# Autodesk Inventor assembly: ASY МОО 001 отстойник осветлитель
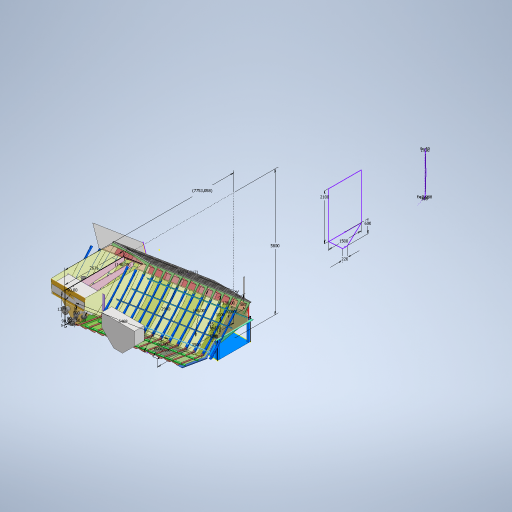
[picture p0: Inventor's stored thumbnail of the model, 512x512]
Saved by Autodesk Inventor 2024.2 (Build 282272000, 272)
## iProperties
Created: 2024-04-28
Part Number: ASY МОО 001 отстойник осветлитель
Document SubType Name: Weldment
Designer: admin
Weld Material: Welded Aluminum-6061
Mass: 1.58517e+06 g
Surface Area: 1.48953e+06 cm^2
Volume: 226523 cm^3
Density: 6.99781 g/cm^3
Author: admin
## Documents named in this file (52)
- C:\Users\admin\YandexDisk-badmisterfox\домашниий пк\Inventor\Manturovo\Manturovo_Se-clar\ASY МОО 001 отстойник осветлитель.iam
- C:\Users\admin\YandexDisk-badmisterfox\домашниий пк\Inventor\Manturovo\Manturovo_Se-clar\МОО 033 лист спина базовый.ipt
- C:\Users\admin\YandexDisk-badmisterfox\домашниий пк\Inventor\Manturovo\Manturovo_Se-clar\Пример емкости.ipt
- C:\Users\admin\YandexDisk-badmisterfox\домашниий пк\Inventor\Manturovo\Manturovo_Se-clar\МОО 041 лист брюхо основной.ipt
- C:\Users\admin\YandexDisk-badmisterfox\домашниий пк\Inventor\Manturovo\Manturovo_Se-clar\МОО 052 шпангоут борт.ipt
- C:\Users\admin\YandexDisk-badmisterfox\домашниий пк\Inventor\Manturovo\Manturovo_Se-clar\МОО 051 шпангоут спина.ipt
- C:\Users\admin\YandexDisk-badmisterfox\домашниий пк\Inventor\Manturovo\Manturovo_Se-clar\Рама основания\ASY МОО 040 рама основания.iam
- C:\Users\admin\YandexDisk-badmisterfox\домашниий пк\Inventor\Manturovo\Manturovo_Se-clar\ASY МОО 060 ракета.iam
- C:\Users\admin\YandexDisk-badmisterfox\домашниий пк\Inventor\Manturovo\Manturovo_Se-clar\Content Center Files\en-US\ISO 5251 B 3D\ISO 5251 Bends 3D without straight ends(90 deg) DN80 2 2.ipt
- C:\Users\admin\YandexDisk-badmisterfox\домашниий пк\Inventor\Manturovo\Manturovo_Se-clar\Content Center Files\en-US\ISO 5251(1)\ISO 5251 Concentric reducers DN80 x DN65 3,2 3,2.ipt
- C:\Users\admin\YandexDisk-badmisterfox\домашниий пк\Inventor\Manturovo\Manturovo_Se-clar\ASY МОО 010 конус.iam
- C:\Users\admin\YandexDisk-badmisterfox\домашниий пк\Inventor\Manturovo\Manturovo_Se-clar\ракета\МОО 064 ракета труба.ipt
- C:\Users\admin\YandexDisk-badmisterfox\домашниий пк\Inventor\Manturovo\Manturovo_Se-clar\х_размеры МОО отстойник осветлитель Dummu.ipt
- C:\Users\admin\YandexDisk-badmisterfox\домашниий пк\Inventor\Manturovo\Manturovo_Se-clar\МОО 031 лист спина поясница.ipt
- C:\Users\admin\YandexDisk-badmisterfox\домашниий пк\Inventor\Manturovo\Manturovo_Se-clar\Content Center Files\en-US\DIN EN 1092-1 01 - PN 25\DIN EN 1092-1 Plate Flange for Welding Type 01 - PN 25 80 x 88.9.ipt
- C:\Users\admin\YandexDisk-badmisterfox\домашниий пк\Inventor\Manturovo\Manturovo_Se-clar\МОО 024 лист борт основной.ipt
- C:\Users\admin\YandexDisk-badmisterfox\домашниий пк\Inventor\Manturovo\Manturovo_Se-clar\МОО 032 лист спина-поясница магич.ipt
- C:\Users\admin\YandexDisk-badmisterfox\домашниий пк\Inventor\Manturovo\Manturovo_Se-clar\МОО 021 лист левый борт бедро.ipt
- C:\Users\admin\YandexDisk-badmisterfox\домашниий пк\Inventor\Manturovo\Manturovo_Se-clar\МОО 022 лист правый борт бедро.ipt
- C:\Users\admin\YandexDisk-badmisterfox\домашниий пк\Inventor\Manturovo\Manturovo_Se-clar\МОО 034 лист спина-холка.ipt
- C:\Users\admin\YandexDisk-badmisterfox\домашниий пк\Inventor\Manturovo\Manturovo_Se-clar\МОО 042 лист брюхо-горло.ipt
- C:\Users\admin\YandexDisk-badmisterfox\домашниий пк\Inventor\Manturovo\Manturovo_Se-clar\МОО 023 лист борт.ipt
- C:\Users\admin\YandexDisk-badmisterfox\домашниий пк\Inventor\Manturovo\Manturovo_Se-clar\конус\МОО 071 гребень 1.ipt
- C:\Users\admin\YandexDisk-badmisterfox\домашниий пк\Inventor\Manturovo\Manturovo_Se-clar\конус\МОО 072 гребень 2.ipt
- C:\Users\admin\YandexDisk-badmisterfox\домашниий пк\Inventor\Manturovo\Manturovo_Se-clar\конус\МОО 073 морда 3.ipt
- C:\Users\admin\YandexDisk-badmisterfox\домашниий пк\Inventor\Manturovo\Manturovo_Se-clar\Content Center Files\en-US\ISO 5251 B 3D\ISO 5251 Bends 3D without straight ends(90 deg) DN150 11 11.ipt
- C:\Users\admin\YandexDisk-badmisterfox\домашниий пк\Inventor\Manturovo\Manturovo_Se-clar\Content Center Files\en-US\DIN EN 1092-1 01 - PN 25\DIN EN 1092-1 Plate Flange for Welding Type 01 - PN 25 150 x 168.3.ipt
- C:\Users\admin\YandexDisk-badmisterfox\домашниий пк\Inventor\Manturovo\Manturovo_Se-clar\МОО 061 труба верх 1.ipt
- C:\Users\admin\YandexDisk-badmisterfox\домашниий пк\Inventor\Manturovo\Manturovo_Se-clar\МОО 062 труба верх 2.ipt
- C:\Users\admin\YandexDisk-badmisterfox\домашниий пк\Inventor\Manturovo\Manturovo_Se-clar\МОО 063 труба верх 3.ipt
- C:\Users\admin\YandexDisk-badmisterfox\домашниий пк\Inventor\Manturovo\Manturovo_Se-clar\МОО 061 стрингер спина ^.ipt
- C:\Users\admin\YandexDisk-badmisterfox\домашниий пк\Inventor\Manturovo\Manturovo_Se-clar\МОО 063 стрингер борт #.ipt
- C:\Users\admin\YandexDisk-badmisterfox\домашниий пк\Inventor\Manturovo\Manturovo_Se-clar\МОО 062 стрингер спина ^^.ipt
- C:\Users\admin\YandexDisk-badmisterfox\домашниий пк\Inventor\Manturovo\Manturovo_Se-clar\МОО 064 стрингер борт ##.ipt
- C:\Users\admin\YandexDisk-badmisterfox\домашниий пк\Inventor\Manturovo\Manturovo_Se-clar\МОО 065 стрингер борт ###.ipt
- C:\Users\admin\YandexDisk-badmisterfox\домашниий пк\Inventor\Manturovo\Manturovo_Se-clar\МОО 066 стрингер борт ####.ipt
- C:\Users\admin\YandexDisk-badmisterfox\домашниий пк\Inventor\Manturovo\Manturovo_Se-clar\МОО 067 стрингер борт живот.ipt
- C:\Users\admin\YandexDisk-badmisterfox\домашниий пк\Inventor\Manturovo\Manturovo_Se-clar\МОО 053 шпангоут брюхо.ipt
- C:\Users\admin\YandexDisk-badmisterfox\домашниий пк\Inventor\Manturovo\Manturovo_Se-clar\МОО 025 лист борт холка.ipt
- C:\Users\admin\YandexDisk-badmisterfox\домашниий пк\Inventor\Manturovo\Manturovo_Se-clar\МОО 026 лист борт морда.ipt
- C:\Users\admin\YandexDisk-badmisterfox\домашниий пк\Inventor\Manturovo\Manturovo_Se-clar\Part1.ipt
- C:\Users\admin\YandexDisk-badmisterfox\домашниий пк\Inventor\Manturovo\Manturovo_Se-clar\стапель\ASY стапель.iam
- C:\Users\admin\YandexDisk-badmisterfox\домашниий пк\Inventor\Manturovo\Manturovo_Se-clar\DXF файлы\Шпангоуты+стрингеры\МОО 0100.ipt
- C:\Users\admin\YandexDisk-badmisterfox\домашниий пк\Inventor\Manturovo\Manturovo_Se-clar\МОО 025 лист борт холка_MIR.ipt
- C:\Users\admin\YandexDisk-badmisterfox\домашниий пк\Inventor\Manturovo\Manturovo_Se-clar\МОО 026 лист борт морда_MIR.ipt
- C:\Users\admin\YandexDisk-badmisterfox\домашниий пк\Inventor\Manturovo\Manturovo_Se-clar\МОО 068 stringer lowerback.ipt
- C:\Users\admin\YandexDisk-badmisterfox\домашниий пк\Inventor\Manturovo\Manturovo_Se-clar\конус\МОО 071 гребень 1_MIR.ipt
- C:\Users\admin\YandexDisk-badmisterfox\домашниий пк\Inventor\Manturovo\Manturovo_Se-clar\Для удаления\DUMMY 2.ipt
- C:\Users\admin\YandexDisk-badmisterfox\домашниий пк\Inventor\Manturovo\Manturovo_Se-clar\MSC 075 face 5.ipt
- C:\Users\admin\YandexDisk-badmisterfox\домашниий пк\Inventor\Manturovo\Manturovo_Se-clar\MSC 075 face 6.ipt
- C:\Users\admin\YandexDisk-badmisterfox\домашниий пк\Inventor\Manturovo\Manturovo_Se-clar\Для удаления\DUMMY 3.ipt
- C:\Users\admin\YandexDisk-badmisterfox\домашниий пк\Inventor\Manturovo\Manturovo_Se-clar\MSC 077 face 7.ipt
## Components (212 placed, 64 different names)
1. Пример емкости.ipt:1 — Mate:1, Mate:2, Flush:2
2. х_размеры МОО отстойник осветлитель Dummu.ipt:1
3. ASY МОО 040 рама основания.iam:1 [sub-assembly] — Flush:19, Flush:20, Flush:21
4. МОО 033 лист спина базовый.ipt:1 — Flush:3, Rigid:11, Rigid:12
5. МОО 041 лист брюхо основной.ipt:1 — Mate:9, Rigid:18, Rigid:40
6. ASY МОО 060 ракета.iam:1 [sub-assembly] — Flush:23, Rigid:10
7. ISO 5251 Bends 3D without straight ends(90 deg) DN80 2 2.ipt:1 — Rigid:2, Rigid:3
8. ISO 5251 Concentric reducers DN80 x DN65 3,2 3,2.ipt:1 — Rigid:2, Rigid:10
9. ASY МОО 010 конус.iam:1 [sub-assembly] — Flush:22, Mate:16, Flush:28, Mate:31, Mate:36, Mate:54, Mate:57, Mate:65
10. МОО 064 ракета труба.ipt:1 — Rigid:3, Cylindrical:1
11. МОО 033 лист спина базовый.ipt:2 — Rigid:11, Tangent:1, Tangent:3, Rigid:37
12. МОО 033 лист спина базовый.ipt:3 — Flush:24, Rigid:12, Mate:19, Mate:22, Rigid:30, Mate:31, Flush:44, Tangent:8, Tangent:9
13. МОО 031 лист спина поясница.ipt:1 — Mate:15, Mate:16, Flush:27, Mate:19, Mate:22, Tangent:10
14. DIN EN 1092-1 Plate Flange for Welding Type 01 - PN 25 80 x 88.9.ipt:1 — Flush:25, Flush:26, Mate:18, Cylindrical:1
15. МОО 024 лист борт основной.ipt:1 — Flush:30, Tangent:1, Rigid:35, Mate:37
16. МОО 041 лист брюхо основной.ipt:2 — Rigid:18, Rigid:53
17. МОО 032 лист спина-поясница магич.ipt:1 — Mate:24, Rigid:30, Flush:42, Tangent:6, Flush:43, Tangent:7
18. МОО 021 лист левый борт бедро.ipt:1 — Flush:41, Flush:42, Tangent:6
19. МОО 022 лист правый борт бедро.ipt:1 — Mate:30, Flush:43, Tangent:7
20. МОО 024 лист борт основной.ipt:2 — Rigid:35, Rigid:36
21. МОО 024 лист борт основной.ipt:3 — Rigid:36, Rigid:49
22. МОО 033 лист спина базовый.ipt:4 — Rigid:37, Rigid:38
23. МОО 033 лист спина базовый.ipt:5 — Rigid:38, Rigid:39
24. МОО 034 лист спина-холка.ipt:1 — Rigid:39
25. МОО 041 лист брюхо основной.ipt:3 — Rigid:40, Rigid:47
26. МОО 042 лист брюхо-горло.ipt:1 — Rigid:48, Mate:70, Mate:71
27. МОО 041 лист брюхо основной.ipt:4 — Rigid:45, Rigid:47
28. МОО 041 лист брюхо основной.ipt:5 — Rigid:45, Rigid:48
29. МОО 024 лист борт основной.ipt:4 — Rigid:49, Rigid:50
30. МОО 024 лист борт основной.ipt:5 — Rigid:50, Rigid:113
31. МОО 023 лист борт.ipt:1 — Mate:36, Flush:47, Tangent:8, Mate:37, Mate:55
32. МОО 071 гребень 1.ipt:1 — Mate:50, Flush:57, Mate:68
33. МОО 073 морда 3.ipt:2 — Rigid:156, Rigid:157, Mate:70, Flush:62, Mate:71, Rigid:159
34. МОО 041 лист брюхо основной.ipt:6 — Mate:54, Mate:55, Rigid:53
35. DIN EN 1092-1 Plate Flange for Welding Type 01 - PN 25 80 x 88.9.ipt:2 — Rigid:62
36. МОО 072 гребень 2.ipt:2 — Flush:56, Flush:57, Mate:68, Flush:59, Mate:77, Flush:78
37. DIN EN 1092-1 Plate Flange for Welding Type 01 - PN 25 150 x 168.3.ipt:1 — Rigid:158
38. МОО 061 труба верх 1.ipt:1 — Rigid:158, Rigid:59, Rigid:159
39. ISO 5251 Bends 3D without straight ends(90 deg) DN150 11 11.ipt:1 — Rigid:59, Rotational:2
40. МОО 062 труба верх 2.ipt:1 — Rigid:132, Rigid:156
41. DIN EN 1092-1 Plate Flange for Welding Type 01 - PN 25 150 x 168.3.ipt:2 — Rigid:132
42. МОО 063 труба верх 3.ipt:1 — Rigid:62, Rigid:157
43. МОО 024 лист борт основной.ipt:6 — Rigid:134
44. МОО 024 лист борт основной.ipt:7
45. МОО 024 лист борт основной.ipt:8
46. МОО 024 лист борт основной.ipt:9
47. МОО 024 лист борт основной.ipt:10 — Rigid:67
48. МОО 023 лист борт.ipt:2 — Rigid:67, Mate:57, Mate:58, Tangent:9
49. МОО 052 шпангоут борт.ipt:1 — Rigid:74, Rigid:128, Rigid:129
50. МОО 051 шпангоут спина.ipt:1 — Rigid:25, Rigid:74, Rigid:91, Rigid:93, Rigid:139
51. МОО 066 стрингер борт ####.ipt:1 — Rigid:143
52. МОО 065 стрингер борт ###.ipt:1 — Rigid:142
53. МОО 064 стрингер борт ##.ipt:1 — Rigid:129, Rigid:141
54. МОО 063 стрингер борт #.ipt:1 — Rigid:128, Rigid:140
55. МОО 062 стрингер спина ^^.ipt:1 — Rigid:93, Rigid:155
56. МОО 061 стрингер спина ^.ipt:2 — Rigid:91, Rigid:153
57. МОО 061 стрингер спина ^.ipt:1 — Rigid:90, Rigid:152
58. МОО 025 лист борт холка.ipt:1 — Rigid:113, Rigid:114
59. МОО 026 лист борт морда.ipt:1 — Rigid:114, Flush:56, Mate:69, Flush:60, Mate:75
60. Part1.ipt:1
61. МОО 051 шпангоут спина.ipt:2 — Rigid:116, Rigid:121, Rigid:130, Rigid:131
62. МОО 051 шпангоут спина.ipt:3 — Rigid:116
63. МОО 051 шпангоут спина.ipt:4 — Rigid:131
64. МОО 051 шпангоут спина.ipt:5 — Mate:62, Flush:53
65. МОО 052 шпангоут борт.ipt:2 — Rigid:121
66. МОО 062 стрингер спина ^^.ipt:2 — Rigid:92, Mate:66, Rigid:154
67. МОО 066 стрингер борт ####.ipt:2 — Rigid:125, Rigid:151
68. МОО 063 стрингер борт #.ipt:2 — Rigid:122, Rigid:148
69. МОО 064 стрингер борт ##.ipt:2 — Rigid:123, Rigid:149
70. МОО 065 стрингер борт ###.ipt:2 — Rigid:124, Rigid:150
71. МОО 052 шпангоут борт.ipt:3 — Rigid:72, Rigid:122, Rigid:123, Flush:51, Flush:52, Rigid:124, Rigid:125, Mate:61
72. МОО 051 шпангоут спина.ipt:6 — Flush:12, Tangent:3, Rigid:25, Flush:44, Rigid:72, Rigid:90, Rigid:92, Rigid:130
73. ASY стапель.iam:1 [sub-assembly] — Mate:62, Flush:53, Mate:63
74. МОО 053 шпангоут брюхо.ipt:2 — Rigid:110, Flush:51, Flush:52, Rigid:126, Mate:61, Rigid:127
75. МОО 053 шпангоут брюхо.ipt:1 — Rigid:111, Rigid:112, Rigid:127
76. МОО 067 стрингер борт живот.ipt:4 — Rigid:126, Rigid:147
77. МОО 067 стрингер борт живот.ipt:3 — Rigid:110, Rigid:146
78. МОО 067 стрингер борт живот.ipt:2 — Rigid:112, Rigid:144
79. МОО 067 стрингер борт живот.ipt:1 — Rigid:111, Rigid:145
80. МОО 0100.ipt:1 — Mate:64
81. МОО 025 лист борт холка_MIR:1 — Rigid:133, Rigid:134
82. МОО 026 лист борт морда_MIR:1 — Rigid:133
83. МОО 068 stringer lowerback:1 — Mate:65, Mate:66, Tangent:10
84. МОО 071 гребень 1_MIR:1 — Flush:58
85. МОО 061 труба верх 1:2 — Rotational:2
86. DUMMY 2:1 — Flush:59
87. MSC 075 face 5:1 — Mate:69, Flush:60, Flush:61, Mate:76
88. MSC 075 face 6:1 — Flush:76, Mate:75, Mate:76
89. DUMMY 3:1
90. DIN EN 1092-1 Plate Flange for Welding Type 01 - PN 25 80 x 88.9:3
91. МОО 063 труба верх 3:2
92. MSC 077 face 7:1 — Mate:77, Flush:77, Flush:78
93. МОО 042 шпангоут брюхо:4
94. МОО 052 шпангоут борт:5
95. МОО 051 шпангоут спина:31 — Rigid:139
96. МОО 051 шпангоут спина:30
97. МОО 052 шпангоут борт:4
98. МОО 042 шпангоут брюхо:3
99. МОО 042 шпангоут брюхо:5
100. МОО 052 шпангоут борт:6
101. МОО 051 шпангоут спина:32
102. МОО 051 шпангоут спина:33
103. МОО 052 шпангоут борт:7
104. МОО 042 шпангоут брюхо:6
105. МОО 042 шпангоут брюхо:7
106. МОО 052 шпангоут борт:8
107. МОО 051 шпангоут спина:34
108. МОО 051 шпангоут спина:35
109. МОО 052 шпангоут борт:9
110. МОО 042 шпангоут брюхо:8
111. МОО 042 шпангоут брюхо:9
112. МОО 052 шпангоут борт:10
113. МОО 051 шпангоут спина:36
114. МОО 051 шпангоут спина:37
115. МОО 052 шпангоут борт:11
116. МОО 042 шпангоут брюхо:10
117. МОО 042 шпангоут брюхо:11
118. МОО 052 шпангоут борт:12
119. МОО 051 шпангоут спина:38
120. МОО 051 шпангоут спина:39
121. МОО 052 шпангоут борт:13
122. МОО 042 шпангоут брюхо:12
123. МОО 042 шпангоут брюхо:13
124. МОО 052 шпангоут борт:14
125. МОО 051 шпангоут спина:40
126. МОО 051 шпангоут спина:41
127. МОО 052 шпангоут борт:15
128. МОО 042 шпангоут брюхо:14
129. МОО 042 шпангоут брюхо:15
130. МОО 052 шпангоут борт:16
131. МОО 051 шпангоут спина:42
132. МОО 051 шпангоут спина:43
133. МОО 052 шпангоут борт:17
134. МОО 042 шпангоут брюхо:16
135. МОО 042 шпангоут брюхо:17
136. МОО 052 шпангоут борт:18
137. МОО 051 шпангоут спина:44
138. МОО 051 шпангоут спина:45
139. МОО 052 шпангоут борт:19
140. МОО 042 шпангоут брюхо:18
141. МОО 042 шпангоут брюхо:19
142. МОО 052 шпангоут борт:20
143. МОО 051 шпангоут спина:46
144. МОО 051 шпангоут спина:47
145. МОО 052 шпангоут борт:21
146. МОО 042 шпангоут брюхо:20
147. МОО 042 шпангоут брюхо:21
148. МОО 052 шпангоут борт:22
149. МОО 051 шпангоут спина:48
150. МОО 051 шпангоут спина:49
151. МОО 052 шпангоут борт:23
152. МОО 042 шпангоут брюхо:22
153. МОО 042 шпангоут брюхо:23
154. МОО 052 шпангоут борт:24
155. МОО 051 шпангоут спина:50
156. МОО 051 шпангоут спина:51
157. МОО 052 шпангоут борт:25
158. МОО 042 шпангоут брюхо:24
159. МОО 042 шпангоут брюхо:25
160. МОО 052 шпангоут борт:26
161. МОО 051 шпангоут спина:52
162. МОО 051 шпангоут спина:53
163. МОО 052 шпангоут борт:27
164. МОО 042 шпангоут брюхо:26
165. МОО 053 стрингер борт 3:4 — Rigid:148
166. МОО 054 стрингер борт 4:4 — Rigid:149
167. МОО 055 стрингер борт 5:4 — Rigid:150
168. МОО 056 стрингер борт 6:4 — Rigid:151
169. МОО 057 стрингер борт 7:5 — Rigid:147
170. МОО 057 стрингер борт 7:6 — Rigid:146
171. МОО 052 стрингер спина 2:4 — Rigid:154
172. МОО 051 стрингер спина 1:4 — Rigid:152
173. МОО 051 стрингер спина 1:3 — Rigid:153
174. МОО 052 стрингер спина 2:3 — Rigid:155
175. МОО 053 стрингер борт 3:3 — Rigid:140
176. МОО 054 стрингер борт 4:3 — Rigid:141
177. МОО 055 стрингер борт 5:3 — Rigid:142
178. МОО 056 стрингер борт 6:3 — Rigid:143
179. МОО 057 стрингер борт 7:10 — Rigid:145
180. МОО 057 стрингер борт 7:9 — Rigid:144
181. МОО 053 стрингер борт 3:5
182. МОО 054 стрингер борт 4:5
183. МОО 055 стрингер борт 5:5
184. МОО 056 стрингер борт 6:5
185. МОО 057 стрингер борт 7:11
186. МОО 057 стрингер борт 7:12
187. МОО 052 стрингер спина 2:5
188. МОО 051 стрингер спина 1:5
189. МОО 051 стрингер спина 1:7
190. МОО 052 стрингер спина 2:7
191. МОО 053 стрингер борт 3:7
192. МОО 054 стрингер борт 4:7
193. МОО 055 стрингер борт 5:7
194. МОО 056 стрингер борт 6:7
195. МОО 057 стрингер борт 7:15
196. МОО 057 стрингер борт 7:17
197. МОО 053 стрингер борт 3:6
198. МОО 054 стрингер борт 4:6
199. МОО 055 стрингер борт 5:6
200. МОО 056 стрингер борт 6:6
201. МОО 057 стрингер борт 7:13
202. МОО 057 стрингер борт 7:14
203. МОО 052 стрингер спина 2:6
204. МОО 051 стрингер спина 1:6
205. МОО 051 стрингер спина 1:8
206. МОО 052 стрингер спина 2:8
207. МОО 053 стрингер борт 3:8
208. МОО 054 стрингер борт 4:8
209. МОО 055 стрингер борт 5:8
210. МОО 056 стрингер борт 6:8
211. МОО 057 стрингер борт 7:16
212. МОО 057 стрингер борт 7:18
## Component patterns: (12 elements, first: МОО 042 шпангоут брюхо:4 + МОО 052 шпангоут борт:5 + МОО 051 шпангоут спина:31 + МОО 051 шпангоут спина:30 + МОО 052 шпангоут борт:4 + МОО 042 шпангоут брюхо:3), (3 elements, first: МОО 053 стрингер борт 3:4 + МОО 054 стрингер борт 4:4 + МОО 055 стрингер борт 5:4 + МОО 056 стрингер борт 6:4 + МОО 057 стрингер борт 7:5 + МОО 057 стрингер борт 7:6 + МОО 052 стрингер спина 2:4 + МОО 051 стрингер спина 1:4 + МОО 051 стрингер спина 1:3 + МОО 052 стрингер спина 2:3 + МОО 053 стрингер борт 3:3 + МОО 054 стрингер борт 4:3 + МОО 055 стрингер борт 5:3 + МОО 056 стрингер борт 6:3 + МОО 057 стрингер борт 7:10 + МОО 057 стрингер борт 7:9)
## Relationships (155: WeldJoint 80, Flush 34, Mate 32, Tangent 7, CylindricalJoint 1, RevoluteJoint 1)
- Mate:1: Пример емкости.ipt:1
- Mate:2: Пример емкости.ipt:1
- Flush:2: Пример емкости.ipt:1
- Flush:3: МОО 033 лист спина базовый.ipt:1
- Mate:9: МОО 041 лист брюхо основной.ipt:1
- Flush:12: МОО 051 шпангоут спина.ipt:6
- Rigid:2 [WeldJoint]: ISO 5251 Bends 3D without straight ends(90 deg) DN80 2 2.ipt:1 ↔ ISO 5251 Concentric reducers DN80 x DN65 3,2 3,2.ipt:1
- Rigid:3 [WeldJoint]: ISO 5251 Bends 3D without straight ends(90 deg) DN80 2 2.ipt:1 ↔ МОО 064 ракета труба.ipt:1
- Flush:19 (-250 mm): ASY МОО 040 рама основания.iam:1
- Flush:20: ASY МОО 040 рама основания.iam:1
- Flush:21: ASY МОО 040 рама основания.iam:1
- Flush:22: ASY МОО 010 конус.iam:1
- Flush:23: ASY МОО 060 ракета.iam:1
- Mate:15: МОО 031 лист спина поясница.ipt:1
- Flush:24: МОО 033 лист спина базовый.ipt:3
- Mate:16: ASY МОО 010 конус.iam:1 ↔ МОО 031 лист спина поясница.ipt:1
- Flush:25: DIN EN 1092-1 Plate Flange for Welding Type 01 - PN 25 80 x 88.9.ipt:1
- Flush:26: DIN EN 1092-1 Plate Flange for Welding Type 01 - PN 25 80 x 88.9.ipt:1
- Mate:18 (120 mm): DIN EN 1092-1 Plate Flange for Welding Type 01 - PN 25 80 x 88.9.ipt:1
- Rigid:10 [WeldJoint] (-20 mm): ASY МОО 060 ракета.iam:1 ↔ ISO 5251 Concentric reducers DN80 x DN65 3,2 3,2.ipt:1
- Cylindrical:1: МОО 064 ракета труба.ipt:1 ↔ DIN EN 1092-1 Plate Flange for Welding Type 01 - PN 25 80 x 88.9.ipt:1
- Flush:27 (15 mm): МОО 031 лист спина поясница.ipt:1
- Flush:28: ASY МОО 010 конус.iam:1
- Rigid:11 [WeldJoint]: МОО 033 лист спина базовый.ipt:1 ↔ МОО 033 лист спина базовый.ipt:2
- Rigid:12 [WeldJoint]: МОО 033 лист спина базовый.ipt:1 ↔ МОО 033 лист спина базовый.ipt:3
- Mate:19 (910 mm): МОО 033 лист спина базовый.ipt:3 ↔ МОО 031 лист спина поясница.ipt:1
- Flush:30: МОО 024 лист борт основной.ipt:1
- Tangent:1: МОО 033 лист спина базовый.ipt:2 ↔ МОО 024 лист борт основной.ipt:1
- Tangent:3: МОО 033 лист спина базовый.ipt:2 ↔ МОО 051 шпангоут спина.ipt:6
- Mate:22 (47 mm): МОО 033 лист спина базовый.ipt:3 ↔ МОО 031 лист спина поясница.ipt:1
- Rigid:18 [WeldJoint]: МОО 041 лист брюхо основной.ipt:1 ↔ МОО 041 лист брюхо основной.ipt:2
- Rigid:25 [WeldJoint] (-50 mm): МОО 051 шпангоут спина.ipt:1 ↔ МОО 051 шпангоут спина.ipt:6
- Mate:24: МОО 032 лист спина-поясница магич.ipt:1
- Rigid:30 [WeldJoint]: МОО 033 лист спина базовый.ipt:3 ↔ МОО 032 лист спина-поясница магич.ipt:1
- Flush:41: МОО 021 лист левый борт бедро.ipt:1
- Flush:42: МОО 032 лист спина-поясница магич.ipt:1 ↔ МОО 021 лист левый борт бедро.ipt:1
- Tangent:6: МОО 032 лист спина-поясница магич.ipt:1 ↔ МОО 021 лист левый борт бедро.ipt:1
- Mate:30: МОО 022 лист правый борт бедро.ipt:1
- Flush:43: МОО 032 лист спина-поясница магич.ipt:1 ↔ МОО 022 лист правый борт бедро.ipt:1
- Tangent:7: МОО 032 лист спина-поясница магич.ipt:1 ↔ МОО 022 лист правый борт бедро.ipt:1
- Rigid:35 [WeldJoint]: МОО 024 лист борт основной.ipt:1 ↔ МОО 024 лист борт основной.ipt:2
- Rigid:36 [WeldJoint]: МОО 024 лист борт основной.ipt:2 ↔ МОО 024 лист борт основной.ipt:3
- Rigid:37 [WeldJoint]: МОО 033 лист спина базовый.ipt:2 ↔ МОО 033 лист спина базовый.ipt:4
- Rigid:38 [WeldJoint]: МОО 033 лист спина базовый.ipt:4 ↔ МОО 033 лист спина базовый.ipt:5
- Rigid:39 [WeldJoint]: МОО 033 лист спина базовый.ipt:5 ↔ МОО 034 лист спина-холка.ipt:1
- Mate:31: ASY МОО 010 конус.iam:1 ↔ МОО 033 лист спина базовый.ipt:3
- Rigid:40 [WeldJoint]: МОО 041 лист брюхо основной.ipt:1 ↔ МОО 041 лист брюхо основной.ipt:3
- Flush:44 (-250 mm): МОО 033 лист спина базовый.ipt:3 ↔ МОО 051 шпангоут спина.ipt:6
- Rigid:45 [WeldJoint]: МОО 041 лист брюхо основной.ipt:4 ↔ МОО 041 лист брюхо основной.ipt:5
- Rigid:47 [WeldJoint]: МОО 041 лист брюхо основной.ipt:3 ↔ МОО 041 лист брюхо основной.ipt:4
- Rigid:48 [WeldJoint]: МОО 042 лист брюхо-горло.ipt:1 ↔ МОО 041 лист брюхо основной.ipt:5
- Rigid:49 [WeldJoint]: МОО 024 лист борт основной.ipt:3 ↔ МОО 024 лист борт основной.ipt:4
- Rigid:50 [WeldJoint]: МОО 024 лист борт основной.ipt:4 ↔ МОО 024 лист борт основной.ipt:5
- Mate:36: ASY МОО 010 конус.iam:1 ↔ МОО 023 лист борт.ipt:1
- Flush:47: МОО 023 лист борт.ipt:1
- Tangent:8: МОО 033 лист спина базовый.ipt:3 ↔ МОО 023 лист борт.ipt:1
- Mate:37: МОО 024 лист борт основной.ipt:1 ↔ МОО 023 лист борт.ipt:1
- Mate:50 (200 mm): МОО 071 гребень 1.ipt:1
- Mate:54: ASY МОО 010 конус.iam:1 ↔ МОО 041 лист брюхо основной.ipt:6
- Mate:55: МОО 023 лист борт.ipt:1 ↔ МОО 041 лист брюхо основной.ipt:6
- Rigid:53 [WeldJoint]: МОО 041 лист брюхо основной.ipt:2 ↔ МОО 041 лист брюхо основной.ipt:6
- Rigid:158 [WeldJoint]: DIN EN 1092-1 Plate Flange for Welding Type 01 - PN 25 150 x 168.3.ipt:1 ↔ МОО 061 труба верх 1.ipt:1
- Rigid:59 [WeldJoint]: МОО 061 труба верх 1.ipt:1 ↔ ISO 5251 Bends 3D without straight ends(90 deg) DN150 11 11.ipt:1
- Rigid:62 [WeldJoint]: DIN EN 1092-1 Plate Flange for Welding Type 01 - PN 25 80 x 88.9.ipt:2 ↔ МОО 063 труба верх 3.ipt:1
- [WeldJoint]: МОО 024 лист борт основной.ipt:6 ↔ МОО 024 лист борт основной.ipt:7
- [WeldJoint]: МОО 024 лист борт основной.ipt:7 ↔ МОО 024 лист борт основной.ipt:8
- [WeldJoint]: МОО 024 лист борт основной.ipt:8 ↔ МОО 024 лист борт основной.ipt:9
- [WeldJoint]: МОО 024 лист борт основной.ipt:9 ↔ МОО 024 лист борт основной.ipt:10
- Rigid:67 [WeldJoint]: МОО 024 лист борт основной.ipt:10 ↔ МОО 023 лист борт.ipt:2
- Mate:57: ASY МОО 010 конус.iam:1 ↔ МОО 023 лист борт.ipt:2
- Mate:58: МОО 023 лист борт.ipt:2
- Tangent:9: МОО 033 лист спина базовый.ipt:3 ↔ МОО 023 лист борт.ipt:2
- Rigid:72 [WeldJoint] (-50 mm): МОО 052 шпангоут борт.ipt:3 ↔ МОО 051 шпангоут спина.ipt:6
- Rigid:74 [WeldJoint] (-50 mm): МОО 052 шпангоут борт.ipt:1 ↔ МОО 051 шпангоут спина.ipt:1
- Rigid:90 [WeldJoint] (2 mm): МОО 061 стрингер спина ^.ipt:1 ↔ МОО 051 шпангоут спина.ipt:6
- Rigid:91 [WeldJoint] (2 mm): МОО 051 шпангоут спина.ipt:1 ↔ МОО 061 стрингер спина ^.ipt:2
- Rigid:92 [WeldJoint] (2 mm): МОО 062 стрингер спина ^^.ipt:2 ↔ МОО 051 шпангоут спина.ipt:6
- Rigid:93 [WeldJoint] (2 mm): МОО 051 шпангоут спина.ipt:1 ↔ МОО 062 стрингер спина ^^.ipt:1
- Rigid:110 [WeldJoint] (2 mm): МОО 053 шпангоут брюхо.ipt:2 ↔ МОО 067 стрингер борт живот.ipt:3
- Rigid:111 [WeldJoint] (2 mm): МОО 053 шпангоут брюхо.ipt:1 ↔ МОО 067 стрингер борт живот.ipt:1
- Rigid:112 [WeldJoint] (2 mm): МОО 053 шпангоут брюхо.ipt:1 ↔ МОО 067 стрингер борт живот.ipt:2
- Rigid:113 [WeldJoint]: МОО 024 лист борт основной.ipt:5 ↔ МОО 025 лист борт холка.ipt:1
- Rigid:114 [WeldJoint]: МОО 025 лист борт холка.ipt:1 ↔ МОО 026 лист борт морда.ipt:1
- Rigid:116 [WeldJoint] (50 mm): МОО 051 шпангоут спина.ipt:2 ↔ МОО 051 шпангоут спина.ipt:3
- [WeldJoint] (50 mm): МОО 051 шпангоут спина.ipt:4 ↔ МОО 051 шпангоут спина.ipt:5
- Rigid:121 [WeldJoint] (-50 mm): МОО 051 шпангоут спина.ipt:2 ↔ МОО 052 шпангоут борт.ipt:2
- Rigid:122 [WeldJoint] (2 mm): МОО 063 стрингер борт #.ipt:2 ↔ МОО 052 шпангоут борт.ipt:3
- Rigid:123 [WeldJoint] (2 mm): МОО 064 стрингер борт ##.ipt:2 ↔ МОО 052 шпангоут борт.ipt:3
- Flush:51: МОО 052 шпангоут борт.ipt:3 ↔ МОО 053 шпангоут брюхо.ipt:2
- Flush:52: МОО 052 шпангоут борт.ipt:3 ↔ МОО 053 шпангоут брюхо.ipt:2
- Rigid:124 [WeldJoint] (2 mm): МОО 065 стрингер борт ###.ipt:2 ↔ МОО 052 шпангоут борт.ipt:3
- Rigid:125 [WeldJoint]: МОО 066 стрингер борт ####.ipt:2 ↔ МОО 052 шпангоут борт.ipt:3
- Rigid:126 [WeldJoint] (2 mm): МОО 053 шпангоут брюхо.ipt:2 ↔ МОО 067 стрингер борт живот.ipt:4
- Mate:61: МОО 052 шпангоут борт.ipt:3 ↔ МОО 053 шпангоут брюхо.ipt:2
- Mate:62: МОО 051 шпангоут спина.ipt:5 ↔ ASY стапель.iam:1
- Flush:53: МОО 051 шпангоут спина.ipt:5 ↔ ASY стапель.iam:1
- Mate:63: ASY стапель.iam:1
- Rigid:127 [WeldJoint] (-50 mm): МОО 053 шпангоут брюхо.ipt:2 ↔ МОО 053 шпангоут брюхо.ipt:1
- Rigid:128 [WeldJoint] (2 mm): МОО 052 шпангоут борт.ipt:1 ↔ МОО 063 стрингер борт #.ipt:1
- Rigid:129 [WeldJoint] (2 mm): МОО 052 шпангоут борт.ipt:1 ↔ МОО 064 стрингер борт ##.ipt:1
- Rigid:130 [WeldJoint] (-500 mm): МОО 051 шпангоут спина.ipt:2 ↔ МОО 051 шпангоут спина.ipt:6
- Rigid:131 [WeldJoint] (-500 mm): МОО 051 шпангоут спина.ipt:2 ↔ МОО 051 шпангоут спина.ipt:4
- Rigid:132 [WeldJoint]: МОО 062 труба верх 2.ipt:1 ↔ DIN EN 1092-1 Plate Flange for Welding Type 01 - PN 25 150 x 168.3.ipt:2
- Mate:64: МОО 0100.ipt:1
- Rigid:133 [WeldJoint]: МОО 025 лист борт холка_MIR:1 ↔ МОО 026 лист борт морда_MIR:1
- Rigid:134 [WeldJoint]: МОО 024 лист борт основной.ipt:6 ↔ МОО 025 лист борт холка_MIR:1
- Mate:65: ASY МОО 010 конус.iam:1 ↔ МОО 068 stringer lowerback:1
- Mate:66: МОО 062 стрингер спина ^^.ipt:2 ↔ МОО 068 stringer lowerback:1
- Tangent:10: МОО 031 лист спина поясница.ipt:1 ↔ МОО 068 stringer lowerback:1
- [WeldJoint] (-50 mm): МОО 051 шпангоут спина:31 ↔ МОО 051 шпангоут спина:30
- [WeldJoint] (-50 mm): МОО 051 шпангоут спина:30 ↔ МОО 052 шпангоут борт:4
- [WeldJoint] (-50 mm): МОО 052 шпангоут борт:5 ↔ МОО 051 шпангоут спина:31
- [Flush]: МОО 052 шпангоут борт:4 ↔ МОО 042 шпангоут брюхо:3
- [Flush]: МОО 052 шпангоут борт:4 ↔ МОО 042 шпангоут брюхо:3
- [Mate]: МОО 052 шпангоут борт:4 ↔ МОО 042 шпангоут брюхо:3
- [WeldJoint] (-50 mm): МОО 042 шпангоут брюхо:4 ↔ МОО 042 шпангоут брюхо:3
- Rigid:139 [WeldJoint] (-500 mm): МОО 051 шпангоут спина.ipt:1 ↔ МОО 051 шпангоут спина:31
- Rigid:140 [WeldJoint]: МОО 063 стрингер борт #.ipt:1 ↔ МОО 053 стрингер борт 3:3
- Rigid:141 [WeldJoint]: МОО 064 стрингер борт ##.ipt:1 ↔ МОО 054 стрингер борт 4:3
- Rigid:142 [WeldJoint]: МОО 065 стрингер борт ###.ipt:1 ↔ МОО 055 стрингер борт 5:3
- Rigid:143 [WeldJoint]: МОО 066 стрингер борт ####.ipt:1 ↔ МОО 056 стрингер борт 6:3
- Rigid:144 [WeldJoint]: МОО 067 стрингер борт живот.ipt:2 ↔ МОО 057 стрингер борт 7:9
- Rigid:145 [WeldJoint]: МОО 067 стрингер борт живот.ipt:1 ↔ МОО 057 стрингер борт 7:10
- Rigid:146 [WeldJoint]: МОО 067 стрингер борт живот.ipt:3 ↔ МОО 057 стрингер борт 7:6
- Rigid:147 [WeldJoint]: МОО 067 стрингер борт живот.ipt:4 ↔ МОО 057 стрингер борт 7:5
- Rigid:148 [WeldJoint]: МОО 063 стрингер борт #.ipt:2 ↔ МОО 053 стрингер борт 3:4
- Rigid:149 [WeldJoint]: МОО 064 стрингер борт ##.ipt:2 ↔ МОО 054 стрингер борт 4:4
- Rigid:150 [WeldJoint]: МОО 065 стрингер борт ###.ipt:2 ↔ МОО 055 стрингер борт 5:4
- Rigid:151 [WeldJoint]: МОО 066 стрингер борт ####.ipt:2 ↔ МОО 056 стрингер борт 6:4
- Rigid:152 [WeldJoint]: МОО 061 стрингер спина ^.ipt:1 ↔ МОО 051 стрингер спина 1:4
- Rigid:153 [WeldJoint]: МОО 061 стрингер спина ^.ipt:2 ↔ МОО 051 стрингер спина 1:3
- Rigid:154 [WeldJoint]: МОО 062 стрингер спина ^^.ipt:2 ↔ МОО 052 стрингер спина 2:4
- Rigid:155 [WeldJoint]: МОО 062 стрингер спина ^^.ipt:1 ↔ МОО 052 стрингер спина 2:3
- Flush:56 (200 mm): МОО 072 гребень 2.ipt:2 ↔ МОО 026 лист борт морда.ipt:1
- Flush:57: МОО 071 гребень 1.ipt:1 ↔ МОО 072 гребень 2.ipt:2
- Mate:68: МОО 071 гребень 1.ipt:1 ↔ МОО 072 гребень 2.ipt:2
- Flush:58 (200 mm): МОО 071 гребень 1_MIR:1
- Rotational:2 [RevoluteJoint]: ISO 5251 Bends 3D without straight ends(90 deg) DN150 11 11.ipt:1 ↔ МОО 061 труба верх 1:2
- Flush:59: МОО 072 гребень 2.ipt:2 ↔ DUMMY 2:1
- Mate:69: МОО 026 лист борт морда.ipt:1 ↔ MSC 075 face 5:1
- Flush:60: МОО 026 лист борт морда.ipt:1 ↔ MSC 075 face 5:1
- Flush:61: MSC 075 face 5:1
- Rigid:156 [WeldJoint]: МОО 073 морда 3.ipt:2 ↔ МОО 062 труба верх 2.ipt:1
- Rigid:157 [WeldJoint]: МОО 073 морда 3.ipt:2 ↔ МОО 063 труба верх 3.ipt:1
- Mate:70: МОО 042 лист брюхо-горло.ipt:1 ↔ МОО 073 морда 3.ipt:2
- Flush:62: МОО 073 морда 3.ipt:2
- Mate:71: МОО 042 лист брюхо-горло.ipt:1 ↔ МОО 073 морда 3.ipt:2
- Rigid:159 [WeldJoint] (-200 mm): МОО 073 морда 3.ipt:2 ↔ МОО 061 труба верх 1.ipt:1
- Flush:76: MSC 075 face 6:1
- Mate:75: МОО 026 лист борт морда.ipt:1 ↔ MSC 075 face 6:1
- Mate:76: MSC 075 face 5:1 ↔ MSC 075 face 6:1
- [WeldJoint]: DIN EN 1092-1 Plate Flange for Welding Type 01 - PN 25 80 x 88.9:3 ↔ МОО 063 труба верх 3:2
- Mate:77: МОО 072 гребень 2.ipt:2 ↔ MSC 077 face 7:1
- Flush:77: MSC 077 face 7:1
- Flush:78: МОО 072 гребень 2.ipt:2 ↔ MSC 077 face 7:1
## Named parameters: Бак_нахлест_фланца = 25 mm, d230_d194 = 0 mm, d231_d195 = 0 mm, d232_d160 = 0 mm, d233_d161 = 0 mm, d322_d320 = 50 mm, d384_d346 = 0 mm, d385_d359 = -50 mm, d386_d341 = 0 mm, d387_d342 = 0 mm, d388_d243 = -50 mm, d389_d246 = -50 mm, d390_d128 = -50 mm, d445_d225 = 0 mm
